# Autodesk Inventor assembly: 4463570 DHAS-ME-H9-80
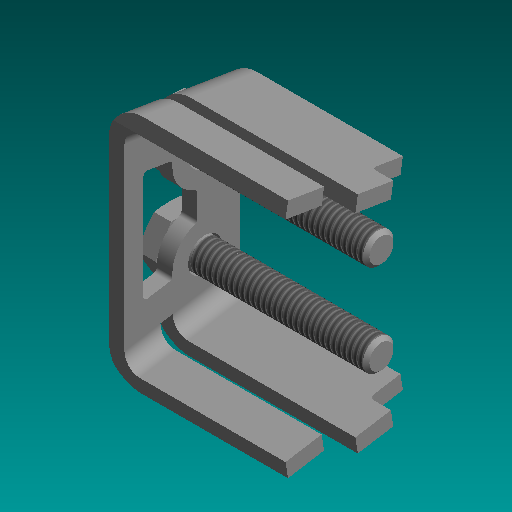
[picture p0: Inventor's stored thumbnail of the model, 512x512]
Saved by Autodesk Inventor 2020.3 (Build 243373000, 373)
## iProperties
Part Number: 4463570 DHAS-ME-H9-80
Catalog Web Link: www.cadenas.de
Description: DHAS-ME-mounting kit
Vendor: FESTO
Document SubType Name: Assembly
Designer: partserver
Manufacturer: FESTO
Mass: 13 g
Surface Area: 33.5387 cm^2
Volume: 2.61227 cm^3
Density: 4.97651 g/cm^3
Category: PARTsolutions
Company: FESTO
PSOL_IDENT_0: {ATYP=ASSISTANT},{DATA=script=$CADENAS_DATA/23d-libs/festo/webfesto.vbb/&M_FAMILY=DHAS&M_GROUP=01&M_
PSOL_IDENT_1: PARTNO=4463570&IDCODE1=DHAS-ME-H9-80&IDCODE2=&customer_number_cns=&MATES=1&LOD=HI&LOCKERP=0&SINGLEPA
PSOL_IDENT_2: RT=1}
NB: 4463570 DHAS-ME-H9-80
NN: DHAS-ME
NT: mounting kit
NBSYN: $TNR. $TYP.
LINA: 4463570 DHAS-ME-H9-80
CATALOG: Festo
TNR: 4463570
TYP: DHAS-ME-H9-80
CNSMASSEXACT: 0.013
SUPPLIER: FESTO
ARTICLENO: 4463570 DHAS-ME-H9-80
BOMINFO: 4463570 DHAS-ME-H9-80
CREATOR: CADENAS GmbH
Title: 4463570 DHAS-ME-H9-80
Author: Cadenas PARTsolutions
Comments: mounting kit
## Documents named in this file (3)
- C:\Users\Svend\OneDrive\Documents\GitHub\BeerMinder\3D-model\servo\AIS2020\4463570 DHAS-ME-H9-80.iam
- C:\Users\Svend\OneDrive\Documents\GitHub\BeerMinder\3D-model\servo\AIS2020\4463570 DHAS-ME-H9-80---(befestigung).ipt
- C:\Users\Svend\OneDrive\Documents\GitHub\BeerMinder\3D-model\servo\AIS2020\Hexagon bolt DIN 933 - M4x25.ipt
## Components (3 placed, 2 different names)
1. 4463570 DHAS-ME-H9-80---(befestigung):1 — DIN933_1_XY@1 <-> IP1_XY@2, DIN933_1_Z@1 <-> IP1_Z@2, DIN933_1_YZ@1 <-> IP1_YZ@2, DIN933_2_XY@1 <-> IP1_XY@3, DIN933_2_Z@1 <-> IP1_Z@3, DIN933_2_YZ@1 <-> IP1_YZ@3
2. Hexagon bolt DIN 933 - M4x25:1 — DIN933_1_XY@1 <-> IP1_XY@2, DIN933_1_Z@1 <-> IP1_Z@2, DIN933_1_YZ@1 <-> IP1_YZ@2
3. Hexagon bolt DIN 933 - M4x25:2 — DIN933_2_XY@1 <-> IP1_XY@3, DIN933_2_Z@1 <-> IP1_Z@3, DIN933_2_YZ@1 <-> IP1_YZ@3
## Relationships (6: Flush 2, Mate 2, Angle 2)
- DIN933_1_XY@1 <-> IP1_XY@2 [Flush]: 4463570 DHAS-ME-H9-80---(befestigung):1 ↔ Hexagon bolt DIN 933 - M4x25:1
- DIN933_1_Z@1 <-> IP1_Z@2 [Mate]: 4463570 DHAS-ME-H9-80---(befestigung):1 ↔ Hexagon bolt DIN 933 - M4x25:1
- DIN933_1_YZ@1 <-> IP1_YZ@2 [Angle] (0 deg): 4463570 DHAS-ME-H9-80---(befestigung):1 ↔ Hexagon bolt DIN 933 - M4x25:1
- DIN933_2_XY@1 <-> IP1_XY@3 [Flush]: 4463570 DHAS-ME-H9-80---(befestigung):1 ↔ Hexagon bolt DIN 933 - M4x25:2
- DIN933_2_Z@1 <-> IP1_Z@3 [Mate]: 4463570 DHAS-ME-H9-80---(befestigung):1 ↔ Hexagon bolt DIN 933 - M4x25:2
- DIN933_2_YZ@1 <-> IP1_YZ@3 [Angle] (0 deg): 4463570 DHAS-ME-H9-80---(befestigung):1 ↔ Hexagon bolt DIN 933 - M4x25:2
